# Autodesk Inventor assembly: Bản vẽ mô tả 3D
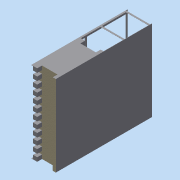
[picture p0: Inventor's stored thumbnail of the model, 180x180]
Saved by Autodesk Inventor 2018 (Build 220112000, 112)
## iProperties
Created: 2020-10-11
Part Number: Bản vẽ mô tả 3D
Document SubType Name: Assembly
Designer: ASUS
Author: ASUS
## Documents named in this file (13)
- E:\CTU\Skylight\Bản vẽ\Bản vẽ Giếng Trời Tự Động\Bản vẽ 3D\Bản vẽ mô tả 3D.iam
- E:\CTU\Skylight\Bản vẽ\Bản vẽ Giếng Trời Tự Động\Bản vẽ 3D\Khung cửa\Khung đỡ.ipt
- E:\CTU\Skylight\Bản vẽ\Bản vẽ Giếng Trời Tự Động\Bản vẽ 3D\Linh kiện khác\Ròng rọc\ròng rọc.iam
- E:\CTU\Skylight\Bản vẽ\Bản vẽ Giếng Trời Tự Động\Bản vẽ 3D\Khung cửa\Khung cửa.ipt
- E:\CTU\Skylight\Bản vẽ\Bản vẽ Giếng Trời Tự Động\Bản vẽ 3D\Linh kiện khác\Ròng rọc\ròng rọc - Bản 2.iam
- E:\CTU\Skylight\Bản vẽ\Bản vẽ Giếng Trời Tự Động\Bản vẽ 3D\Bản vẽ mô tả 3D - Giá đỡ động cơ.iam
- E:\CTU\Skylight\Bản vẽ\Bản vẽ Giếng Trời Tự Động\Bản vẽ 3D\Linh kiện khác\Dây cáp Inox\Dây inox.ipt
- E:\CTU\Skylight\Bản vẽ\Bản vẽ Giếng Trời Tự Động\Bản vẽ 3D\Linh kiện khác\Ốc tán\Ốc + Chốt giữ.ipt
- E:\CTU\Skylight\Bản vẽ\Bản vẽ Giếng Trời Tự Động\Bản vẽ 3D\Linh kiện khác\Ốc tán\Tán + Chốt giữ.ipt
- E:\CTU\Skylight\Bản vẽ\Bản vẽ Giếng Trời Tự Động\Bản vẽ 3D\Linh kiện khác\Tủ điện\Tủ điện.ipt
- E:\CTU\Skylight\Bản vẽ\Bản vẽ Giếng Trời Tự Động\Bản vẽ 3D\Linh kiện khác\Công tắc hành trình\Giá đỡ 1.ipt
- E:\CTU\Skylight\Bản vẽ\Bản vẽ Giếng Trời Tự Động\Bản vẽ 3D\Linh kiện khác\Công tắc hành trình\CTHT.ipt
- E:\CTU\Skylight\Bản vẽ\Bản vẽ Giếng Trời Tự Động\Bản vẽ 3D\Linh kiện khác\Công tắc hành trình\Giá đỡ CTHT 2.ipt
## Components (13 placed, 12 different names)
1. Khung đỡ:1 — Mate:1, Flush:1, Mate:2, Mate:3, Mate:4, Mate:5, Flush:2, Mate:6, Mate:7, Mate:8, Mate:9, Flush:3, Mate:10, Mate:11, Mate:17, Flush:5, Mate:18, Flush:6, Mate:19, Flush:7, Mate:21, Mate:22, Flush:10
2. Khung cửa:1 — Mate:2, Mate:3, Mate:12, Mate:13, Mate:14, Mate:16
3. ròng rọc:1 [sub-assembly] — Mate:1, Flush:1, Mate:9
4. ròng rọc - Bản 2:1 [sub-assembly] — Mate:4, Mate:5, Flush:2
5. Bản vẽ mô tả 3D - Giá đỡ động cơ:1 [sub-assembly] — Mate:6, Mate:7, Mate:8
6. Dây inox:1 — Flush:3, Mate:10, Mate:11
7. Ốc + Chốt giữ:1 — Mate:12, Mate:13, Mate:14, Mate:15, Flush:4
8. Tán + Chốt giữ:1 — Mate:15, Flush:4, Mate:16
9. Tủ điện:1 — Mate:17, Flush:5, Mate:18
10. Giá đỡ 1:1 — Flush:6, Mate:19, Flush:7, Flush:8, Mate:20, Flush:9
11. Giá đỡ CTHT 2:1 — Mate:21, Mate:22, Flush:10, Flush:11, Mate:23, Flush:12
12. CTHT:1 — Flush:8, Mate:20, Flush:9
13. CTHT:2 — Flush:11, Mate:23, Flush:12
## Relationships (35: Mate 23, Flush 12)
- Mate:1 (5 mm): Khung đỡ:1 ↔ ròng rọc:1
- Flush:1 (30 mm): Khung đỡ:1 ↔ ròng rọc:1
- Mate:2 (5 mm): Khung đỡ:1 ↔ Khung cửa:1
- Mate:3 (10 mm): Khung đỡ:1 ↔ Khung cửa:1
- Mate:4: Khung đỡ:1 ↔ ròng rọc - Bản 2:1
- Mate:5 (5 mm): Khung đỡ:1 ↔ ròng rọc - Bản 2:1
- Flush:2 (30 mm): Khung đỡ:1 ↔ ròng rọc - Bản 2:1
- Mate:6: Khung đỡ:1 ↔ Bản vẽ mô tả 3D - Giá đỡ động cơ:1
- Mate:7 (30 mm): Khung đỡ:1 ↔ Bản vẽ mô tả 3D - Giá đỡ động cơ:1
- Mate:8 (-22 mm): Khung đỡ:1 ↔ Bản vẽ mô tả 3D - Giá đỡ động cơ:1
- Mate:9: Khung đỡ:1 ↔ ròng rọc:1
- Flush:3 (-17 mm): Khung đỡ:1 ↔ Dây inox:1
- Mate:10 (-40 mm): Khung đỡ:1 ↔ Dây inox:1
- Mate:11 (28 mm): Khung đỡ:1 ↔ Dây inox:1
- Mate:12 (39.5 mm): Khung cửa:1 ↔ Ốc + Chốt giữ:1
- Mate:13 (-30 mm): Khung cửa:1 ↔ Ốc + Chốt giữ:1
- Mate:14: Khung cửa:1 ↔ Ốc + Chốt giữ:1
- Mate:15: Ốc + Chốt giữ:1 ↔ Tán + Chốt giữ:1
- Flush:4: Ốc + Chốt giữ:1 ↔ Tán + Chốt giữ:1
- Mate:16: Khung cửa:1 ↔ Tán + Chốt giữ:1
- Mate:17: Khung đỡ:1 ↔ Tủ điện:1
- Flush:5 (200 mm): Khung đỡ:1 ↔ Tủ điện:1
- Mate:18 (120 mm): Khung đỡ:1 ↔ Tủ điện:1
- Flush:6 (-1.2 mm): Khung đỡ:1 ↔ Giá đỡ 1:1
- Mate:19: Khung đỡ:1 ↔ Giá đỡ 1:1
- Flush:7: Khung đỡ:1 ↔ Giá đỡ 1:1
- Flush:8: Giá đỡ 1:1 ↔ CTHT:1
- Mate:20: Giá đỡ 1:1 ↔ CTHT:1
- Flush:9: Giá đỡ 1:1 ↔ CTHT:1
- Mate:21: Khung đỡ:1 ↔ Giá đỡ CTHT 2:1
- Mate:22 (30 mm): Khung đỡ:1 ↔ Giá đỡ CTHT 2:1
- Flush:10 (20 mm): Khung đỡ:1 ↔ Giá đỡ CTHT 2:1
- Flush:11: Giá đỡ CTHT 2:1 ↔ CTHT:2
- Mate:23: Giá đỡ CTHT 2:1 ↔ CTHT:2
- Flush:12: Giá đỡ CTHT 2:1 ↔ CTHT:2
